# Autodesk Inventor assembly: buttonassembly
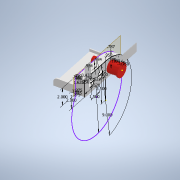
[picture p0: Inventor's stored thumbnail of the model, 180x180]
Saved by Autodesk Inventor 2021 (Build 250183000, 183)
## iProperties
Created: 2020-11-08
Part Number: buttonassembly
Document SubType Name: Assembly
Designer: mackeycj
Author: mackeycj
## Documents named in this file (4)
- C:\Users\mackeycj\Desktop\floorplan2-20201106T152714Z-001\floorplan2\buttonassembly.iam
- C:\Users\mackeycj\Desktop\floorplan2-20201106T152714Z-001\floorplan2\buttonpanel4.5.ipt
- C:\Users\mackeycj\Desktop\floorplan2-20201106T152714Z-001\floorplan2\enclosure.ipt
- C:\Users\mackeycj\Downloads\estop.ipt
## Components (3 placed, 3 different names)
1. buttonpanel4.5:1 — Mate:2, Mate:3, Mate:4, Mate:5, Mate:6
2. enclosure:1 — Mate:1, Mate:2, Mate:3, Mate:4
3. estop:1 — Mate:5, Mate:6
## Relationships (6: Mate 6)
- Mate:1: enclosure:1
- Mate:2: buttonpanel4.5:1 ↔ enclosure:1
- Mate:3: buttonpanel4.5:1 ↔ enclosure:1
- Mate:4: buttonpanel4.5:1 ↔ enclosure:1
- Mate:5: buttonpanel4.5:1 ↔ estop:1
- Mate:6: buttonpanel4.5:1 ↔ estop:1
